# Autodesk Inventor assembly: 조립품1
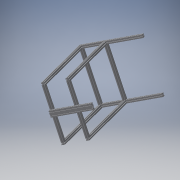
[picture p0: Inventor's stored thumbnail of the model, 180x180]
Saved by Autodesk Inventor 2018 (Build 220112000, 112)
## iProperties
Created: 2020-09-14
Part Number: 조립품1
Material: 일반
Document SubType Name: Assembly
Designer: j3jjj
Author: j3jjj
## Documents named in this file (11)
- C:\Users\j3jjj\Desktop\전자과 캡스톤\3D_응력계산\조립품1.iam
- C:\Users\j3jjj\Desktop\전자과 캡스톤\3D_응력계산\3030600.ipt
- C:\Users\j3jjj\Desktop\전자과 캡스톤\3D_응력계산\3030500.ipt
- C:\Users\j3jjj\Desktop\전자과 캡스톤\3D_응력계산\3030800.ipt
- C:\Users\j3jjj\Desktop\전자과 캡스톤\3D_응력계산\3060400.ipt
- C:\Users\j3jjj\Desktop\전자과 캡스톤\3D_응력계산\조립품1\AIP\FEA\dd3b0rqxs.fins
- C:\Users\j3jjj\Desktop\전자과 캡스톤\3D_응력계산\조립품1\AIP\FEA\dd3b0rqxs.fsat
- C:\Users\j3jjj\Desktop\전자과 캡스톤\3D_응력계산\조립품1\AIP\FEA\dd3b0rqxs.ftes
- C:\Users\j3jjj\Desktop\전자과 캡스톤\3D_응력계산\조립품1\AIP\FEA\dd3b0rqxs.fwiz
- C:\Users\j3jjj\Desktop\전자과 캡스톤\3D_응력계산\조립품1\AIP\FEA\dd3b0rr0g.fmsh
- C:\Users\j3jjj\Desktop\전자과 캡스톤\3D_응력계산\조립품1\AIP\FEA\dd3b0rr0h.fres
## Components (11 placed, 4 different names)
1. 3030600:1 — 메이트:1, 메이트:2, 메이트:3, 메이트:8, 메이트:9, 메이트:12
2. 3030600:2 — 메이트:4, 메이트:5, 메이트:6, 메이트:7, 메이트:10, 메이트:15
3. 3030500:1 — 메이트:1, 메이트:2, 메이트:3, 메이트:4, 메이트:5, 메이트:16
4. 3030800:1 — 메이트:6, 메이트:7, 메이트:11, 메이트:20
5. 3030800:2 — 메이트:10, 메이트:11, 메이트:18, 메이트:19, 메이트:25
6. 3030800:3 — 메이트:8, 메이트:9, 메이트:13, 메이트:21, 메이트:22
7. 3030800:4 — 메이트:12, 메이트:13, 메이트:14, 메이트:17
8. 3030500:2 — 메이트:14, 메이트:15, 메이트:16
9. 3030500:3 — 메이트:17, 메이트:18, 메이트:19, 메이트:24
10. 3030500:4 — 메이트:20, 메이트:21, 메이트:22, 메이트:23
11. 3060400:1 — 메이트:23, 메이트:24, 메이트:25
## Relationships (25: Mate 25)
- 메이트:1 [Mate]: 3030600:1 ↔ 3030500:1
- 메이트:2 [Mate]: 3030600:1 ↔ 3030500:1
- 메이트:3 [Mate]: 3030600:1 ↔ 3030500:1
- 메이트:4 [Mate]: 3030600:2 ↔ 3030500:1
- 메이트:5 [Mate]: 3030600:2 ↔ 3030500:1
- 메이트:6 [Mate]: 3030600:2 ↔ 3030800:1
- 메이트:7 [Mate]: 3030600:2 ↔ 3030800:1
- 메이트:8 [Mate]: 3030600:1 ↔ 3030800:3
- 메이트:9 [Mate]: 3030600:1 ↔ 3030800:3
- 메이트:10 [Mate]: 3030600:2 ↔ 3030800:2
- 메이트:11 [Mate] (200 mm): 3030800:1 ↔ 3030800:2
- 메이트:12 [Mate]: 3030600:1 ↔ 3030800:4
- 메이트:13 [Mate] (200 mm): 3030800:3 ↔ 3030800:4
- 메이트:14 [Mate]: 3030800:4 ↔ 3030500:2
- 메이트:15 [Mate]: 3030600:2 ↔ 3030500:2
- 메이트:16 [Mate] (200 mm): 3030500:1 ↔ 3030500:2
- 메이트:17 [Mate]: 3030800:4 ↔ 3030500:3
- 메이트:18 [Mate]: 3030800:2 ↔ 3030500:3
- 메이트:19 [Mate]: 3030800:2 ↔ 3030500:3
- 메이트:20 [Mate]: 3030800:1 ↔ 3030500:4
- 메이트:21 [Mate]: 3030800:3 ↔ 3030500:4
- 메이트:22 [Mate]: 3030800:3 ↔ 3030500:4
- 메이트:23 [Mate]: 3030500:4 ↔ 3060400:1
- 메이트:24 [Mate]: 3030500:3 ↔ 3060400:1
- 메이트:25 [Mate] (230 mm): 3030800:2 ↔ 3060400:1
## Named parameters: sa_0 = -369.692, sa_1 = 912.102, sa_2 = -177.195
note: some values were not read from the file. Shown as the stored number, unit unknown: "sa_0", "sa_1", "sa_2".
